# Autodesk Inventor assembly: Zusammenbau_Einzelmodul
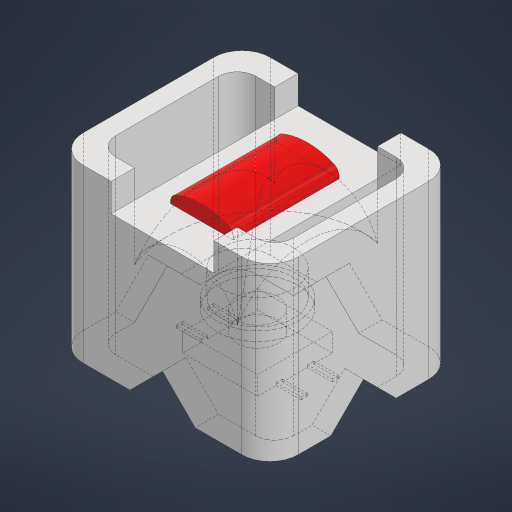
[picture p0: Inventor's stored thumbnail of the model, 512x512]
Saved by Autodesk Inventor 2023 (Build 270158030, 158C)
## iProperties
Created: 2022-05-12
Part Number: Zusammenbau_Einzelmodul
Document SubType Name: Assembly
Designer: Simon
Author: Simon
## Documents named in this file (4)
- C:\Users\simfe\Desktop\2.Semester\Technische Grundlagen-II\Pixie\3d-modelle\.iam's\Zusammenbau_Einzelmodul.iam
- C:\Users\simfe\Desktop\2.Semester\Technische Grundlagen-II\Pixie\3d-modelle\.ipt's\Button.ipt
- C:\Users\simfe\Desktop\2.Semester\Technische Grundlagen-II\Pixie\3d-modelle\.ipt's\LED-streifen.ipt
- C:\Users\simfe\Desktop\2.Semester\Technische Grundlagen-II\Pixie\3d-modelle\.ipt's\Richtfest.ipt
## Components (3 placed, 3 different names)
1. Button:1 — Flush:1
2. LED-streifen:1 — Mate:1
3. Richtfest:1 — Mate:1, Flush:1
## Relationships (2: Mate 1, Flush 1)
- Mate:1: LED-streifen:1 ↔ Richtfest:1
- Flush:1: Button:1 ↔ Richtfest:1
